# Autodesk Inventor assembly: Body Cover Assembly
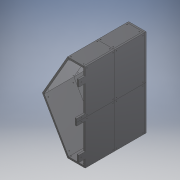
[picture p0: Inventor's stored thumbnail of the model, 180x180]
Saved by Autodesk Inventor 2017 (Build 210142000, 142)
## iProperties
Created: 2018-10-18
Part Number: Body Cover Assembly
Document SubType Name: Assembly
Designer: Dell
Author: Dell
## Documents named in this file (6)
- C:\Users\Dell\Documents\GitHub\tr2\Body\Body Cover Assembly.iam
- C:\Users\Dell\Documents\GitHub\tr2\Body\BO07.ipt
- C:\Users\Dell\Documents\GitHub\tr2\Body\BO08.ipt
- C:\Users\Dell\Documents\GitHub\tr2\Body\BO09.ipt
- C:\Users\Dell\Documents\GitHub\tr2\Body\BO10.ipt
- C:\Users\Dell\Documents\GitHub\tr2\Body\BO11.ipt
## Components (14 placed, 5 different names)
1. BO07:1 — Mate:16, Flush:4, Mate:20, Mate:23
2. BO08:1 — Mate:16, Mate:24
3. BO09:1 — Mate:18, Mate:25
4. BO09:2 — Mate:27
5. BO08:2
6. BO08:3 — Mate:19, Flush:5, Mate:28
7. BO08:4 — Mate:22
8. BO07:2 — Mate:19, Flush:4, Mate:20, Flush:5, Mate:26
9. BO07:3 — Mate:21
10. BO07:4 — Mate:21, Mate:22
11. BO10:1 — Mate:17, Mate:18
12. BO10:2 — Mate:17
13. BO11:1 — Mate:23, Mate:24, Mate:25
14. BO11:2 — Mate:26, Mate:27, Mate:28
## Relationships (33: Mate 28, Flush 5)
- [Mate]: BO09:1 ↔ BO09:2
- [Mate]: BO08:1 ↔ BO09:1
- [Mate]: BO08:1 ↔ BO09:1
- [Mate]: BO07:1 ↔ BO08:1
- [Mate]: BO08:1 ↔ BO08:2
- [Mate]: BO09:1 ↔ BO08:2
- [Mate]: BO09:2 ↔ BO08:3
- [Mate]: BO08:3 ↔ BO08:4
- [Mate]: BO08:3 ↔ BO08:4
- [Mate]: BO07:1 ↔ BO07:2
- [Mate]: BO07:1 ↔ BO07:3
- [Mate]: BO08:2 ↔ BO07:3
- [Mate]: BO07:3 ↔ BO07:4
- [Flush]: BO07:3 ↔ BO07:4
- [Mate]: BO09:2 ↔ BO10:1
- [Flush]: BO09:1 ↔ BO10:1
- [Mate]: BO09:2 ↔ BO10:2
- [Flush]: BO09:2 ↔ BO10:2
- Mate:16: BO07:1 ↔ BO08:1
- Mate:17: BO10:1 ↔ BO10:2
- Mate:18: BO09:1 ↔ BO10:1
- Mate:19: BO08:3 ↔ BO07:2
- Flush:4: BO07:1 ↔ BO07:2
- Mate:20: BO07:1 ↔ BO07:2
- Mate:21: BO07:3 ↔ BO07:4
- Mate:22: BO08:4 ↔ BO07:4
- Flush:5: BO08:3 ↔ BO07:2
- Mate:23: BO07:1 ↔ BO11:1
- Mate:24: BO08:1 ↔ BO11:1
- Mate:25: BO09:1 ↔ BO11:1
- Mate:26: BO07:2 ↔ BO11:2
- Mate:27: BO09:2 ↔ BO11:2
- Mate:28: BO08:3 ↔ BO11:2
